# Autodesk Inventor assembly: portaherramienta
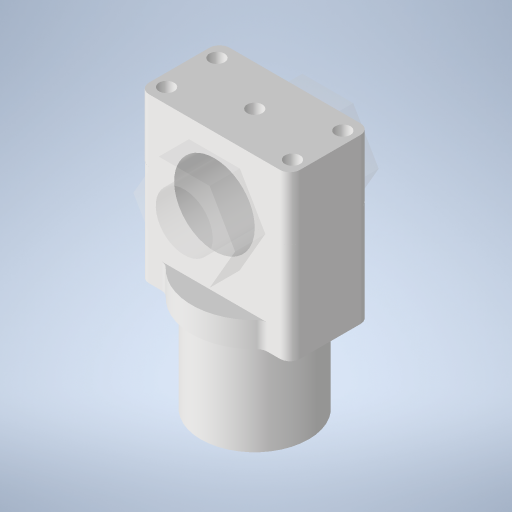
[picture p0: Inventor's stored thumbnail of the model, 512x512]
Saved by Autodesk Inventor 2023 (Build 270158000, 158)
## iProperties
Created: 2022-11-13
Part Number: portaherramienta
Document SubType Name: Assembly
Designer: andre
Author: andre
## Documents named in this file (4)
- C:\Users\andre\Downloads\ProyectoRobotica\CAD\PortaHerramienta\portaherramienta.iam
- C:\Users\andre\Downloads\ProyectoRobotica\CAD\PortaHerramienta\base1.ipt
- C:\Users\andre\Downloads\ProyectoRobotica\CAD\PortaHerramienta\AcopleIntermedio.ipt
- C:\Users\andre\Downloads\ProyectoRobotica\CAD\PortaHerramienta\base2.ipt
## Components (3 placed, 3 different names)
1. base1:1 — Rigid:2, Rigid:3
2. AcopleIntermedio:1 — Rigid:2
3. base2:1 — Rigid:3
## Relationships (2: WeldJoint 2)
- Rigid:2 [WeldJoint]: base1:1 ↔ AcopleIntermedio:1
- Rigid:3 [WeldJoint]: base1:1 ↔ base2:1
